# Autodesk Inventor assembly: support
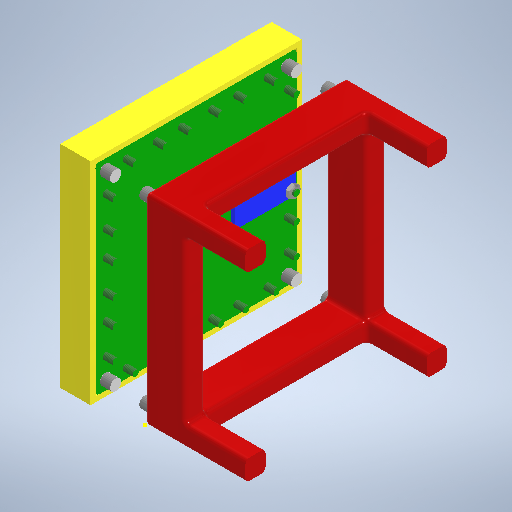
[picture p0: Inventor's stored thumbnail of the model, 512x512]
Saved by Autodesk Inventor 2025.2 (Build 292293000, 293)
## iProperties
Created: 2025-02-15
Part Number: support
Document SubType Name: Assembly
Designer: antoi
Author: antoi
## Documents named in this file (8)
- C:\Users\antoi\Documents\Henallux_24_25\Q2\proj\prototype\support.iam
- C:\Users\antoi\Documents\Henallux_24_25\Q2\proj\prototype\Pièce1.ipt
- C:\Users\antoi\Documents\Henallux_24_25\Q2\proj\prototype\vis.ipt
- C:\Users\antoi\Documents\Henallux_24_25\Q2\proj\prototype\plateau.ipt
- C:\Users\antoi\Documents\Henallux_24_25\Q2\proj\prototype\DFR0440.ipt
- C:\Users\antoi\Documents\Henallux_24_25\Q2\proj\prototype\rebord2.ipt
- C:\Users\antoi\Documents\Henallux_24_25\Q2\proj\prototype\visPlateau.ipt
- C:\Users\antoi\Documents\Inventor\Content Center Files\R2025\fr-FR\ISO 4032(2)\ISO 4032 - M3 - ISO.ipt
## Components (14 placed, 7 different names)
1. Pièce1:1 — Affleurement:1, Placage:1, Placage:2, Placage:3, Placage:4, Affleurement:2, Affleurement:3, Affleurement:4, Affleurement:5
2. vis:1 — Placage:3, Affleurement:2, Placage:5
3. vis:2 — Placage:4, Affleurement:3
4. vis:3 — Placage:2, Affleurement:5, Placage:6
5. vis:4 — Placage:1, Affleurement:4
6. plateau:1 — Placage:5, Placage:6, Placage:7, Placage:8, Placage:14, Placage:15, Placage:16, Placage:17, Placage:18, Placage:19, Placage:20, Affleurement:6, Affleurement:7, Affleurement:8, Affleurement:9, Placage:21, Placage:22, Placage:24
7. DFR0440:1 — Placage:7, Placage:8, Placage:21, Placage:23, Placage:25
8. rebord2:1 — Placage:14, Placage:15, Placage:16
9. visPlateau:1 — Placage:20, Affleurement:6
10. visPlateau:2 — Placage:19, Affleurement:9
11. visPlateau:3 — Placage:18, Affleurement:7
12. visPlateau:4 — Placage:17, Affleurement:8
13. ISO 4032 M3:1 — Placage:24, Placage:25
14. ISO 4032 M3:2 — Placage:22, Placage:23
## Relationships (29: Mate 20, Flush 9)
- Affleurement:1 [Flush] (-5 mm): Pièce1:1
- Placage:1 [Mate]: Pièce1:1 ↔ vis:4
- Placage:2 [Mate]: Pièce1:1 ↔ vis:3
- Placage:3 [Mate]: Pièce1:1 ↔ vis:1
- Placage:4 [Mate]: Pièce1:1 ↔ vis:2
- Affleurement:2 [Flush] (-5 mm): Pièce1:1 ↔ vis:1
- Affleurement:3 [Flush] (-5 mm): Pièce1:1 ↔ vis:2
- Affleurement:4 [Flush] (5 mm): Pièce1:1 ↔ vis:4
- Affleurement:5 [Flush] (-5 mm): Pièce1:1 ↔ vis:3
- Placage:5 [Mate]: vis:1 ↔ plateau:1
- Placage:6 [Mate]: vis:3 ↔ plateau:1
- Placage:7 [Mate]: plateau:1 ↔ DFR0440:1
- Placage:8 [Mate]: plateau:1 ↔ DFR0440:1
- Placage:14 [Mate]: plateau:1 ↔ rebord2:1
- Placage:15 [Mate]: plateau:1 ↔ rebord2:1
- Placage:16 [Mate]: plateau:1 ↔ rebord2:1
- Placage:17 [Mate]: plateau:1 ↔ visPlateau:4
- Placage:18 [Mate]: plateau:1 ↔ visPlateau:3
- Placage:19 [Mate]: plateau:1 ↔ visPlateau:2
- Placage:20 [Mate]: plateau:1 ↔ visPlateau:1
- Affleurement:6 [Flush] (-5 mm): plateau:1 ↔ visPlateau:1
- Affleurement:7 [Flush] (5 mm): plateau:1 ↔ visPlateau:3
- Affleurement:8 [Flush] (-5 mm): plateau:1 ↔ visPlateau:4
- Affleurement:9 [Flush] (5 mm): plateau:1 ↔ visPlateau:2
- Placage:21 [Mate]: plateau:1 ↔ DFR0440:1
- Placage:22 [Mate]: plateau:1 ↔ ISO 4032 M3:2
- Placage:23 [Mate]: DFR0440:1 ↔ ISO 4032 M3:2
- Placage:24 [Mate]: plateau:1 ↔ ISO 4032 M3:1
- Placage:25 [Mate]: DFR0440:1 ↔ ISO 4032 M3:1
